# Autodesk Inventor assembly: mg996r_left_foot_frame
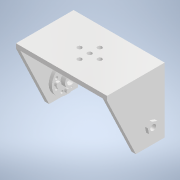
[picture p0: Inventor's stored thumbnail of the model, 180x180]
Saved by Autodesk Inventor 2021.4 (Build 254397000, 397)
## iProperties
Created: 2022-07-25
Part Number: mg996r_left_foot_frame
Document SubType Name: Assembly
Designer: isamu
Author: isamu
## Documents named in this file (6)
- D:\personal_projects\robot\inventor\2021_matlab_compat\mg996r_left_foot_frame.iam
- D:\personal_projects\robot\exports\frames\servo frame mg996 foot.ipt
- D:\personal_projects\robot\exports\handle\servo handle 4.ipt
- D:\personal_projects\robot\exports\screws\m2x8.ipt
- D:\personal_projects\robot\exports\screws\m2 nuts.ipt
- D:\personal_projects\robot\exports\screws\m4 nuts.ipt
## Components (11 placed, 5 different names)
1. servo frame mg996 foot:1 — Mate:1, Mate:2, Mate:3, Insert:5, Insert:6, Insert:7, Insert:8, Insert:10
2. servo handle 4:1 — Mate:1, Mate:2, Mate:3, Insert:1, Insert:2, Insert:3, Insert:4
3. m2x8:1 — Insert:1
4. m2x8:2 — Insert:2
5. m2x8:3 — Insert:3
6. m2x8:4 — Insert:4
7. m2 nuts:1 — Insert:5
8. m2 nuts:2 — Insert:6
9. m2 nuts:3 — Insert:7
10. m2 nuts:4 — Insert:8
11. m4 nuts:1 — Insert:10
## Relationships (12: Insert 9, Mate 3)
- Mate:1: servo frame mg996 foot:1 ↔ servo handle 4:1
- Mate:2: servo frame mg996 foot:1 ↔ servo handle 4:1
- Mate:3: servo frame mg996 foot:1 ↔ servo handle 4:1
- Insert:1: servo handle 4:1 ↔ m2x8:1
- Insert:2: servo handle 4:1 ↔ m2x8:2
- Insert:3: servo handle 4:1 ↔ m2x8:3
- Insert:4: servo handle 4:1 ↔ m2x8:4
- Insert:5: servo frame mg996 foot:1 ↔ m2 nuts:1
- Insert:6: servo frame mg996 foot:1 ↔ m2 nuts:2
- Insert:7: servo frame mg996 foot:1 ↔ m2 nuts:3
- Insert:8: servo frame mg996 foot:1 ↔ m2 nuts:4
- Insert:10: servo frame mg996 foot:1 ↔ m4 nuts:1
